# Autodesk Inventor assembly: Mould20x20
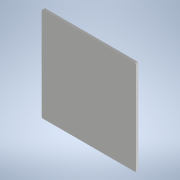
[picture p0: Inventor's stored thumbnail of the model, 180x180]
Saved by Autodesk Inventor 2020 (Build 240168000, 168)
## iProperties
Created: 2020-10-26
Part Number: Mould20x20
Document SubType Name: Assembly
Designer: Naude Conradie
Author: Naude Conradie
## Documents named in this file (4)
- C:\Users\19673418\Documents\Masters-Project\Models\Inventor\Unit Mould\Mould20x20.iam
- C:\Users\19673418\Documents\Masters-Project\Models\Inventor\Unit Mould\MouldBase20x20.ipt
- C:\Users\19673418\Documents\Masters-Project\Models\Inventor\Unit Mould\MouldCellSmall.ipt
- C:\Users\19673418\Documents\Masters-Project\Models\Inventor\Unit Mould\MouldCellLarge.ipt
## Components (3 placed, 3 different names)
1. MouldBase20x20:1 — Mate:10, Mate:11, Mate:12, Mate:13, Mate:14
2. MouldCellSmall:1 — Mate:10, Mate:11, Mate:12, Mate:15
3. MouldCellLarge:1 — Mate:13, Mate:14, Mate:15
## Relationships (6: Mate 6)
- Mate:10: MouldBase20x20:1 ↔ MouldCellSmall:1
- Mate:11: MouldBase20x20:1 ↔ MouldCellSmall:1
- Mate:12: MouldBase20x20:1 ↔ MouldCellSmall:1
- Mate:13: MouldBase20x20:1 ↔ MouldCellLarge:1
- Mate:14: MouldBase20x20:1 ↔ MouldCellLarge:1
- Mate:15: MouldCellSmall:1 ↔ MouldCellLarge:1
